# Autodesk Inventor assembly: BackLink
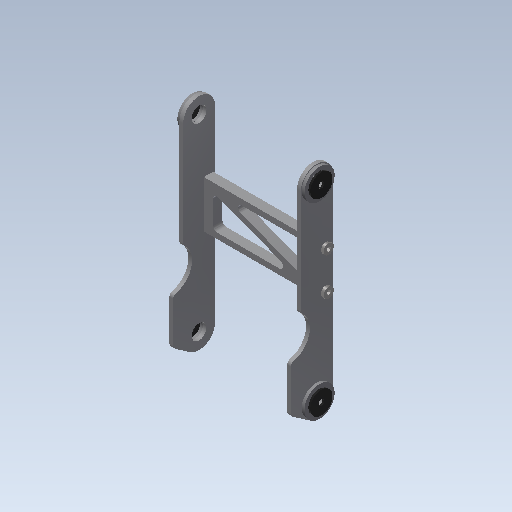
[picture p0: Inventor's stored thumbnail of the model, 512x512]
Saved by Autodesk Inventor 2020.4 (Build 244396000, 396)
## iProperties
Created: 2016-08-23
Part Number: BackLink
Material: 一般
Document SubType Name: Assembly
Designer: hiro
Mass: 27.0677 g
Surface Area: 148.123 cm^2
Volume: 12.1706 cm^3
Density: 2.22402 g/cm^3
Author: hiro
## Documents named in this file (6)
- C:\Users\Masato\Documents\Inventor\CIT Brains_Inventor\OpenPlatform_ver3_0\LowerBody\Link\BackLink.iam
- C:\Users\Masato\Documents\Inventor\CIT Brains_Inventor\OpenPlatform_ver3_0\LowerBody\Link\BackLink_diagonal.ipt
- C:\Users\Masato\Documents\Inventor\CIT Brains_Inventor\OpenPlatform_ver3_0\Ready_Made\UUW-0312-10BH.ipt
- C:\Users\Masato\Documents\Inventor\CIT Brains_Inventor\OpenPlatform_ver3_0\Ready_Made\LFW-0815.ipt
- C:\Users\Masato\Documents\Inventor\CIT Brains_Inventor\OpenPlatform_ver3_0\Ready_Made\Screw\M3-6.ipt
- C:\Users\Masato\Documents\Inventor\CIT Brains_Inventor\OpenPlatform_ver3_0\LowerBody\Link\BackLink_frame.ipt
## Components (15 placed, 5 different names)
1. UUW-0312-10BH:1 — 挿入:30
2. UUW-0312-10BH:2 — 挿入:29
3. UUW-0312-10BH:3 — 挿入:20
4. UUW-0312-10BH:4 — 挿入:19
5. LFW-0815:1 — 挿入:20, 挿入:36
6. LFW-0815:2 — 挿入:19, 挿入:42
7. BackLink_diagonal:1 — 挿入:31, 挿入:32, 挿入:33, 挿入:34, フラッシュ:1, メイト:1
8. LFW-0815:3 — 挿入:29, 挿入:35
9. LFW-0815:4 — 挿入:30, 挿入:39
10. M3-6:1 — 挿入:38
11. M3-6:2 — 挿入:37
12. M3-6:3 — 挿入:41
13. M3-6:4 — 挿入:40
14. BackLink_frame:1 — 挿入:33, 挿入:34, 挿入:35, 挿入:36, 挿入:37, 挿入:38
15. BackLink_frame:2 — 挿入:31, 挿入:32, 挿入:39, 挿入:40, 挿入:41, 挿入:42, フラッシュ:2
## Relationships (19: Insert 16, Flush 2, Mate 1)
- 挿入:19 [Insert]: UUW-0312-10BH:4 ↔ LFW-0815:2
- 挿入:20 [Insert]: UUW-0312-10BH:3 ↔ LFW-0815:1
- 挿入:29 [Insert]: UUW-0312-10BH:2 ↔ LFW-0815:3
- 挿入:30 [Insert]: UUW-0312-10BH:1 ↔ LFW-0815:4
- 挿入:31 [Insert]: BackLink_diagonal:1 ↔ BackLink_frame:2
- 挿入:32 [Insert]: BackLink_diagonal:1 ↔ BackLink_frame:2
- 挿入:33 [Insert]: BackLink_diagonal:1 ↔ BackLink_frame:1
- 挿入:34 [Insert]: BackLink_diagonal:1 ↔ BackLink_frame:1
- 挿入:35 [Insert]: LFW-0815:3 ↔ BackLink_frame:1
- 挿入:36 [Insert]: LFW-0815:1 ↔ BackLink_frame:1
- 挿入:37 [Insert]: M3-6:2 ↔ BackLink_frame:1
- 挿入:38 [Insert]: M3-6:1 ↔ BackLink_frame:1
- 挿入:39 [Insert]: LFW-0815:4 ↔ BackLink_frame:2
- 挿入:40 [Insert]: M3-6:4 ↔ BackLink_frame:2
- 挿入:41 [Insert]: M3-6:3 ↔ BackLink_frame:2
- 挿入:42 [Insert]: LFW-0815:2 ↔ BackLink_frame:2
- フラッシュ:1 [Flush]: BackLink_diagonal:1
- メイト:1 [Mate]: BackLink_diagonal:1
- フラッシュ:2 [Flush]: BackLink_frame:2
